# Autodesk Inventor assembly: hubjig
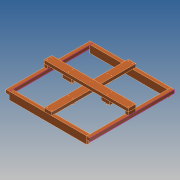
[picture p0: Inventor's stored thumbnail of the model, 180x180]
Saved by Autodesk Inventor 2014 SP1 (Build 180222100, 222)
## iProperties
Created: 2014-08-29
Part Number: hubjig
Document SubType Name: Assembly
Designer: Dave
Author: Dave
## Documents named in this file (7)
- C:\Users\Dave\Desktop\hera-cad\jigs\hubjig.iam
- C:\Users\Dave\Desktop\hera-cad\jigs\hubjig_side1.ipt
- C:\Users\Dave\Desktop\hera-cad\jigs\hubjig_side2.ipt
- C:\Users\Dave\Desktop\hera-cad\jigs\hubjig_cross.ipt
- C:\Users\Dave\Desktop\hera-cad\jigs\hubjig_spacer.ipt
- C:\Users\Dave\Desktop\hera-cad\jigs\hubjig_block.ipt
- C:\Users\Dave\Desktop\hera-cad\jigs\hubjig_tab.ipt
## Components (14 placed, 6 different names)
1. hubjig_side1:1 — Insert:1, Insert:2, Flush:2, Flush:3, Insert:6, Flush:6, Angle:2
2. hubjig_side2:1 — Insert:1, Insert:3, Flush:2, Flush:4
3. hubjig_side2:2 — Insert:2, Insert:4, Flush:1, Flush:3
4. hubjig_side1:2 — Insert:3, Flush:4, Insert:5, Flush:5
5. hubjig_cross:1 — Insert:4, Flush:1, Insert:10, Angle:1, Insert:11, Angle:3
6. hubjig_spacer:1 — Insert:5, Flush:5
7. hubjig_spacer:2 — Insert:6, Flush:6, Insert:7, Flush:7
8. hubjig_cross:2 — Insert:7, Flush:7, Insert:8, Insert:9, Flush:8, Flush:9
9. hubjig_block:1 — Insert:8, Flush:8, Insert:12, Angle:4
10. hubjig_block:2 — Insert:9, Flush:9, Insert:13, Angle:5
11. hubjig_tab:1 — Insert:10, Angle:1
12. hubjig_tab:2 — Insert:11, Angle:3
13. hubjig_tab:3 — Insert:12, Angle:4
14. hubjig_tab:4 — Insert:13, Angle:5
## Relationships (27: Insert 13, Flush 9, Angle 5)
- Insert:1: hubjig_side1:1 ↔ hubjig_side2:1
- Insert:2: hubjig_side1:1 ↔ hubjig_side2:2
- Insert:3: hubjig_side2:1 ↔ hubjig_side1:2
- Insert:4: hubjig_side2:2 ↔ hubjig_cross:1
- Flush:1: hubjig_side2:2 ↔ hubjig_cross:1
- Flush:2: hubjig_side1:1 ↔ hubjig_side2:1
- Flush:3: hubjig_side1:1 ↔ hubjig_side2:2
- Flush:4: hubjig_side2:1 ↔ hubjig_side1:2
- Insert:5: hubjig_side1:2 ↔ hubjig_spacer:1
- Insert:6: hubjig_side1:1 ↔ hubjig_spacer:2
- Flush:5: hubjig_side1:2 ↔ hubjig_spacer:1
- Flush:6: hubjig_side1:1 ↔ hubjig_spacer:2
- Insert:7: hubjig_spacer:2 ↔ hubjig_cross:2
- Flush:7: hubjig_spacer:2 ↔ hubjig_cross:2
- Insert:8: hubjig_cross:2 ↔ hubjig_block:1
- Insert:9: hubjig_cross:2 ↔ hubjig_block:2
- Flush:8: hubjig_cross:2 ↔ hubjig_block:1
- Flush:9: hubjig_cross:2 ↔ hubjig_block:2
- Insert:10: hubjig_cross:1 ↔ hubjig_tab:1
- Angle:1 (180 deg): hubjig_cross:1 ↔ hubjig_tab:1
- Angle:2 (0 deg): hubjig_side1:1
- Insert:11: hubjig_cross:1 ↔ hubjig_tab:2
- Insert:12: hubjig_block:1 ↔ hubjig_tab:3
- Insert:13: hubjig_block:2 ↔ hubjig_tab:4
- Angle:3 (180 deg): hubjig_cross:1 ↔ hubjig_tab:2
- Angle:4 (180 deg): hubjig_block:1 ↔ hubjig_tab:3
- Angle:5 (0 deg): hubjig_block:2 ↔ hubjig_tab:4
